# Autodesk Inventor assembly: 組合2
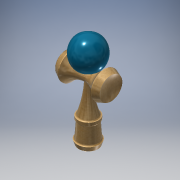
[picture p0: Inventor's stored thumbnail of the model, 180x180]
Saved by Autodesk Inventor 2017 (Build 210142000, 142)
## iProperties
Part Number: 組合2
Material: 一般
Document SubType Name: Assembly
Designer: user
Author: user
## Documents named in this file (4)
- D:\410571040\組合2.iam
- C:\Users\user\Desktop\A.ipt
- C:\Users\user\Desktop\B.ipt
- C:\Users\user\Desktop\C.ipt
## Components (3 placed, 3 different names)
1. A:1 — 貼合:1
2. B:1 — 貼合:1, 插入:1
3. C:1 — 插入:1
## Relationships (2: Mate 1, Insert 1)
- 貼合:1 [Mate]: A:1 ↔ B:1
- 插入:1 [Insert] (30 mm): B:1 ↔ C:1
